# Autodesk Inventor assembly: gearbox4_assembly
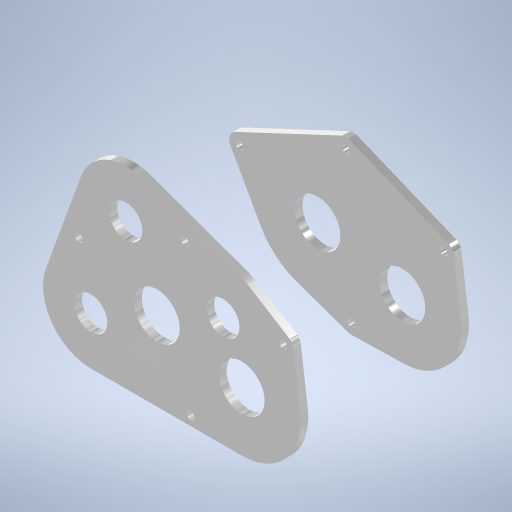
[picture p0: Inventor's stored thumbnail of the model, 512x512]
Saved by Autodesk Inventor 2024 (Build 280153000, 153)
## iProperties
Created: 2024-12-29
Part Number: gearbox4_assembly
Document SubType Name: Assembly
Designer: Danielle
Author: Danielle
## Documents named in this file (3)
- C:\Users\micha\OneDrive\Documents\GitHub\1622-2024-Assignments\Danielle\gearbox 4\gearbox 4 stuff\gearbox4_assembly.iam
- C:\Users\micha\OneDrive\Documents\GitHub\1622-2024-Assignments\Danielle\gearbox 4\gearbox 4 stuff\bottomplate_gearbox4.ipt
- C:\Users\micha\OneDrive\Documents\GitHub\1622-2024-Assignments\Danielle\gearbox 4\gearbox 4 stuff\topplate_gearbox4_trust.ipt
## Components (2 placed, 2 different names)
1. bottomplate_gearbox4:1 — Mate:1, Mate:2, Mate:3
2. topplate_gearbox4_trust:1 — Mate:1, Mate:2, Mate:3
## Relationships (3: Mate 3)
- Mate:1: bottomplate_gearbox4:1 ↔ topplate_gearbox4_trust:1
- Mate:2: bottomplate_gearbox4:1 ↔ topplate_gearbox4_trust:1
- Mate:3: bottomplate_gearbox4:1 ↔ topplate_gearbox4_trust:1
